# Autodesk Inventor assembly: Samenstl Waterkanon poging 1
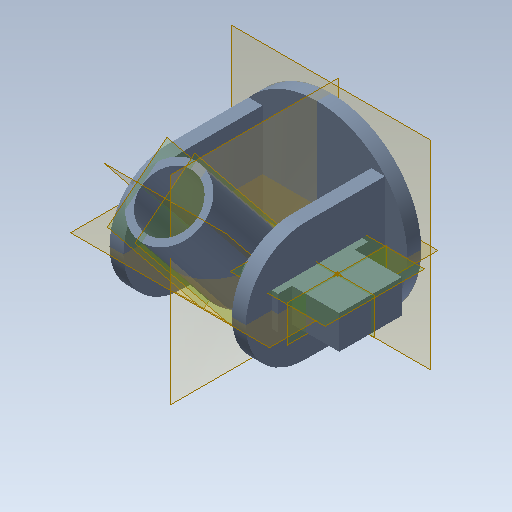
[picture p0: Inventor's stored thumbnail of the model, 512x512]
Saved by Autodesk Inventor 2021 (Build 250183000, 183)
## iProperties
Manager: Pierloot J.
Company: Emmaüs Bovenbouw Aalter
Created: 2017-06-09
Part Number: Samenstl Waterkanon poging 1
Catalog Web Link: http://emmausbovenbouw.op-weg.be/
Vendor: Emmaüs Bovenbouw Aalter
Document SubType Name: Assembly
Designer: declercqs
Engineer: Declercq St.
Authority: Declercq St.
Title: Algemene Projecttitel
Author: declercqs
## Documents named in this file (4)
- C:\Users\Antho\Documents\Inventor\Samenstl Waterkanon poging 1.iam
- C:\Users\Antho\Documents\Inventor\Draaischijf waterkanon poging 2.0.ipt
- C:\Users\Antho\Documents\Inventor\Waterkanon.ipt
- C:\Users\Antho\Documents\Inventor\Motor Waterkanon.ipt
## Components (3 placed, 3 different names)
1. Draaischijf waterkanon poging 2.0:1 — Mate:1, Mate:2, Mate:3, Mate:4
2. Waterkanon:1 — Mate:1, Mate:5
3. Motor Waterkanon:1 — Mate:2, Mate:3, Mate:4, Mate:5
## Relationships (5: Mate 5)
- Mate:1: Draaischijf waterkanon poging 2.0:1 ↔ Waterkanon:1
- Mate:2: Draaischijf waterkanon poging 2.0:1 ↔ Motor Waterkanon:1
- Mate:3: Draaischijf waterkanon poging 2.0:1 ↔ Motor Waterkanon:1
- Mate:4: Draaischijf waterkanon poging 2.0:1 ↔ Motor Waterkanon:1
- Mate:5: Waterkanon:1 ↔ Motor Waterkanon:1
